# Autodesk Inventor assembly: Assembly1
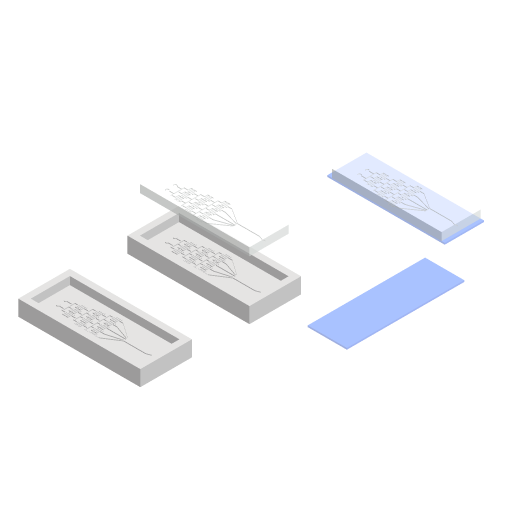
[picture p0: Inventor's stored thumbnail of the model, 512x512]
Saved by Autodesk Inventor 2023 (Build 270158000, 158)
## iProperties
Created: 2022-09-28
Part Number: Assembly1
Document SubType Name: Assembly
Designer: ferrerx
Author: ferrerx
## Documents named in this file (4)
- C:\Users\ferrerx\Documents\GitHub\Four_channel_syringe_pump\Gradient chip\Assembly1.iam
- C:\Users\ferrerx\Documents\GitHub\Four_channel_syringe_pump\Gradient chip\Microfluidics gradient PDMS.ipt
- C:\Users\ferrerx\Documents\GitHub\Four_channel_syringe_pump\Gradient chip\Microfluidics gradient.ipt
- C:\Users\ferrerx\Documents\GitHub\Four_channel_syringe_pump\Gradient chip\Microscope slide.ipt
## Components (6 placed, 3 different names)
1. Microfluidics gradient PDMS:1 — Mate:1, Mate:2
2. Microfluidics gradient:1 — Flush:5, Flush:8
3. Microscope slide:1 — Flush:4, Mate:3, Flush:6, Flush:7
4. Microfluidics gradient PDMS:2 — Flush:4, Mate:3, Flush:7
5. Microfluidics gradient:2 — Mate:1, Mate:2, Flush:5, Flush:6, Flush:8
6. Microscope slide:2
## Relationships (8: Flush 5, Mate 3)
- Mate:1: Microfluidics gradient PDMS:1 ↔ Microfluidics gradient:2
- Mate:2: Microfluidics gradient PDMS:1 ↔ Microfluidics gradient:2
- Flush:4: Microscope slide:1 ↔ Microfluidics gradient PDMS:2
- Mate:3: Microscope slide:1 ↔ Microfluidics gradient PDMS:2
- Flush:5: Microfluidics gradient:1 ↔ Microfluidics gradient:2
- Flush:6: Microscope slide:1 ↔ Microfluidics gradient:2
- Flush:7 (-2 mm): Microscope slide:1 ↔ Microfluidics gradient PDMS:2
- Flush:8: Microfluidics gradient:1 ↔ Microfluidics gradient:2
